# Autodesk Inventor assembly: Neck Support
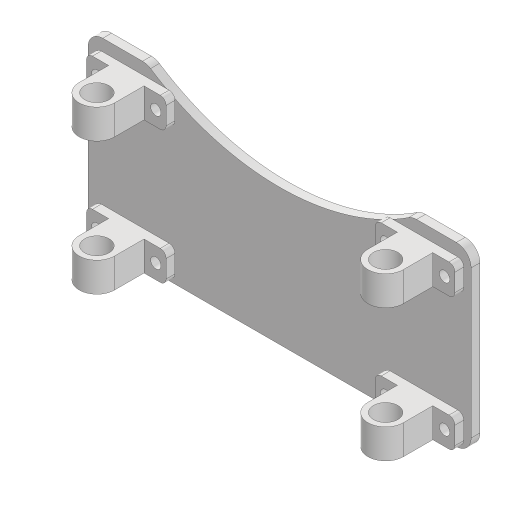
[picture p0: Inventor's stored thumbnail of the model, 512x512]
Saved by Autodesk Inventor 2024 (Build 280153000, 153)
## iProperties
Created: 2025-04-26
Part Number: Neck Support
Document SubType Name: Assembly
Designer: Binara
Author: Binara
## Documents named in this file (3)
- Z:\Robotics\Inventor\Auto Chair\Neck Support\Neck Support.iam
- Z:\Robotics\Inventor\Auto Chair\Neck Support\Base plate.ipt
- Z:\Robotics\Inventor\Auto Chair\Neck Support\Rod Holder.ipt
## Components (5 placed, 2 different names)
1. Base plate:1 — Mate:1, Rigid:2, Rigid:1, Rigid:3, Rigid:4
2. Rod Holder:1 — Mate:1, Rigid:2
3. Rod Holder:2 — Rigid:1
4. Rod Holder:3 — Rigid:3
5. Rod Holder:4 — Rigid:4
## Relationships (5: WeldJoint 4, Mate 1)
- Mate:1: Base plate:1 ↔ Rod Holder:1
- Rigid:2 [WeldJoint]: Base plate:1 ↔ Rod Holder:1
- Rigid:1 [WeldJoint]: Base plate:1 ↔ Rod Holder:2
- Rigid:3 [WeldJoint]: Base plate:1 ↔ Rod Holder:3
- Rigid:4 [WeldJoint]: Base plate:1 ↔ Rod Holder:4
